# Autodesk Inventor assembly: A2017_T5_05
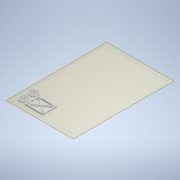
[picture p0: Inventor's stored thumbnail of the model, 180x180]
Saved by Autodesk Inventor 2020 (Build 240168000, 168)
## iProperties
Created: 2021-08-27
Part Number: A2017_T5_05
Document SubType Name: Assembly
Designer: Masato
Author: Masato
## Documents named in this file (4)
- C:\Inventor\SUSTAINA-OP\Cam\A2017_T5_06.iam
- C:\Inventor\SUSTAINA-OP\Cam\DisposableBoard.ipt
- C:\Inventor\SUSTAINA-OP\UpperBody\Trunk\CrossRollerBearing\Inner_support_stand.ipt
- C:\Inventor\SUSTAINA-OP\LowerBody\Link\FrontLink_diagonal.ipt
## Components (4 placed, 3 different names)
1. DisposableBoard:1 — メイト:2, メイト:1, フラッシュ:1, フラッシュ:2, メイト:20, 角度:4, 正接:1, 正接:2, メイト:22, フラッシュ:5
2. FrontLink_diagonal:1 — メイト:22, 正接:16, フラッシュ:5
3. Inner_support_stand:1 — メイト:20, 角度:4, 正接:1, 正接:2
4. Inner_support_stand:2 — 正接:16
## Component patterns: (2 elements, first: Inner_support_stand:1)
## Relationships (11: Mate 4, Flush 3, Tangent 3, Angle 1)
- メイト:2 [Mate]: DisposableBoard:1
- メイト:1 [Mate]: DisposableBoard:1
- フラッシュ:1 [Flush]: DisposableBoard:1
- フラッシュ:2 [Flush]: DisposableBoard:1
- メイト:20 [Mate]: DisposableBoard:1 ↔ Inner_support_stand:1
- 角度:4 [Angle] (0 deg): DisposableBoard:1 ↔ Inner_support_stand:1
- 正接:1 [Tangent] (2 mm): DisposableBoard:1 ↔ Inner_support_stand:1
- 正接:2 [Tangent] (2 mm): DisposableBoard:1 ↔ Inner_support_stand:1
- メイト:22 [Mate]: DisposableBoard:1 ↔ FrontLink_diagonal:1
- 正接:16 [Tangent] (2.5 mm): FrontLink_diagonal:1 ↔ Inner_support_stand:2
- フラッシュ:5 [Flush] (2 mm): DisposableBoard:1 ↔ FrontLink_diagonal:1
